# Autodesk Inventor assembly: outsideHand
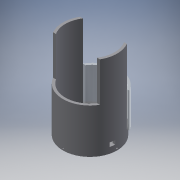
[picture p0: Inventor's stored thumbnail of the model, 180x180]
Saved by Autodesk Inventor 2016 (Build 200138000, 138)
## iProperties
Created: 2016-11-10
Part Number: outsideHand
Material: 一般
Document SubType Name: Assembly
Designer: Daisuke
Author: Daisuke
## Documents named in this file (5)
- C:\Users\Daisuke\Documents\GitHub\CAD\Hand\ver1\outsideHand.iam
- C:\Users\Daisuke\Documents\GitHub\CAD\Hand\ver1\outsideBottom.ipt
- C:\Users\Daisuke\Documents\GitHub\CAD\Hand\ver1\UFL08 -Housing.ipt
- C:\Users\Daisuke\Documents\GitHub\CAD\Hand\ver1\outsideCover.iam
- C:\Users\Daisuke\Documents\GitHub\CAD\Hand\ver1\outsideCover1.ipt
## Components (4 placed, 4 different names)
1. outsideBottom:1 — 挿入:2, 挿入:3, 挿入:4, メイト:1, メイト:2, 挿入:5
2. UFL08 -Housing:1 — 挿入:2, 挿入:3
3. outsideCover:1 [sub-assembly] — 挿入:4, メイト:1
4. outsideCover1:1 — メイト:2, 挿入:5
## Relationships (6: Insert 4, Mate 2)
- 挿入:2 [Insert]: outsideBottom:1 ↔ UFL08 -Housing:1
- 挿入:3 [Insert]: outsideBottom:1 ↔ UFL08 -Housing:1
- 挿入:4 [Insert]: outsideBottom:1 ↔ outsideCover:1
- メイト:1 [Mate]: outsideBottom:1 ↔ outsideCover:1
- メイト:2 [Mate]: outsideBottom:1 ↔ outsideCover1:1
- 挿入:5 [Insert]: outsideBottom:1 ↔ outsideCover1:1
